# Autodesk Inventor assembly: Assembly_Cube_RMS_Objective_Holder_v3
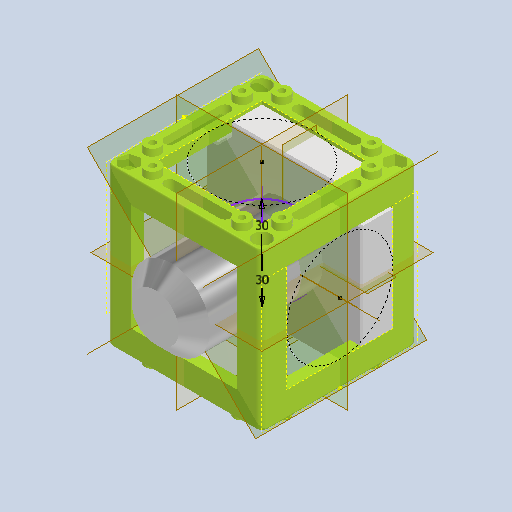
[picture p0: Inventor's stored thumbnail of the model, 512x512]
Saved by Autodesk Inventor 2022 (Build 260153000, 153)
## iProperties
Created: 2022-09-23
Part Number: Assembly_Cube_RMS_Objective_Holder_v3
Document SubType Name: Assembly
Designer: eda_b
Author: eda_b
## Documents named in this file (4)
- G:\My Drive\ASP - M.Sc. Photonics\Practical Modules\MODULE 4 - Master Thesis\2.Experiments\Modules\9.Adjustable_Z_Stage_Module\Assembly_Cube_RMS_Objective_Holder_v3.iam
- G:\My Drive\ASP - M.Sc. Photonics\Practical Modules\MODULE 4 - Master Thesis\2.Experiments\Modules\2.Base_Cube\Base_Cube_IM\Assembly_Cube_empty_IM_v3.iam
- G:\My Drive\ASP - M.Sc. Photonics\Practical Modules\MODULE 4 - Master Thesis\2.Experiments\Modules\9.Adjustable_Z_Stage_Module\Manually_driven_MGN12H_Z_Stage\00_Microscope_Objective_Lens10x.ipt
- G:\My Drive\ASP - M.Sc. Photonics\Practical Modules\MODULE 4 - Master Thesis\2.Experiments\Modules\9.Adjustable_Z_Stage_Module\20_Cube_Insert_RMS.ipt
## Components (3 placed, 3 different names)
1. Assembly_Cube_empty_IM_v3:1 [sub-assembly] — Mate:1, Flush:1, Flush:2
2. 00_Microscope_Objective_Lens10x:1 — Rotational:1
3. 20_Cube_Insert_RMS:1 — Mate:1, Flush:1, Flush:2, Rotational:1
## Relationships (4: Flush 2, Mate 1, RevoluteJoint 1)
- Mate:1: Assembly_Cube_empty_IM_v3:1 ↔ 20_Cube_Insert_RMS:1
- Flush:1: Assembly_Cube_empty_IM_v3:1 ↔ 20_Cube_Insert_RMS:1
- Flush:2: Assembly_Cube_empty_IM_v3:1 ↔ 20_Cube_Insert_RMS:1
- Rotational:1 [RevoluteJoint]: 00_Microscope_Objective_Lens10x:1 ↔ 20_Cube_Insert_RMS:1
